# Autodesk Inventor assembly: Lift 3
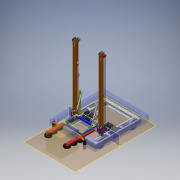
[picture p0: Inventor's stored thumbnail of the model, 180x180]
Saved by Autodesk Inventor 2017 SP1 (Build 210196100, 196)
## iProperties
Created: 2018-01-18
Part Number: Lift 3
Document SubType Name: Assembly
Designer: Ben
Mass: 9979.66 g
Surface Area: 70095.8 cm^2
Volume: 103427 cm^3
Density: 0.0964899 g/cm^3
Author: Ben
## Documents named in this file (23)
- C:\Users\Ben\Desktop\Projects\2018 Robot\Cube Lift\Lift 3.iam
- C:\Users\Ben\Desktop\Projects\2018 Robot\Cube Lift\Rail.ipt
- C:\Users\Ben\Desktop\Projects\2018 Robot\Chassis\2018_chassis.iam
- C:\Users\Ben\Desktop\Projects\2018 Robot\Cube Lift\roller bushing.iam
- C:\Users\Ben\Desktop\Projects\2018 Robot\Cube Lift\cube.ipt
- C:\Users\Ben\Desktop\Projects\2018 Robot\Cube Lift\carriage plate square 2.ipt
- C:\Users\Ben\Desktop\Projects\2018 Robot\Cube Lift\support plate 2.ipt
- C:\Users\Ben\Desktop\Projects\2018 Robot\Cube Lift\top pully bracket.ipt
- C:\Users\Ben\Desktop\Projects\2018 Robot\Cube Lift\pulley XL 1in.ipt
- C:\Users\Ben\Desktop\Projects\2018 Robot\Cube Lift\pulley XL 1.375in 2.ipt
- C:\Users\Ben\Desktop\Projects\2018 Robot\Cube Lift\first stage belt.ipt
- C:\Users\Ben\Desktop\Projects\2018 Robot\Cube Lift\upper anchor.ipt
- C:\Users\Ben\Desktop\Projects\2018 Robot\Cube Lift\top pully bracket 2.ipt
- C:\Users\Ben\Desktop\Projects\2018 Robot\Cube Lift\second stage belt 2.ipt
- C:\Users\Ben\Desktop\Projects\2018 Robot\Cube Lift\carriage plate for intake.ipt
- C:\Users\Ben\Desktop\Projects\2018 Robot\Cube Intake\Intake 2.iam
- C:\Users\Ben\Desktop\Projects\2018 Robot\Cube Lift\cylinder arm.ipt
- C:\Users\Ben\Desktop\Projects\2018 Robot\Cube Lift\cylinder body.ipt
- C:\Users\Ben\Desktop\Projects\2018 Robot\Cube Lift\cylinder piston.ipt
- C:\Users\Ben\Desktop\Projects\2018 Robot\Cube Lift\line pulley.ipt
- C:\Users\Ben\Desktop\Projects\2018 Robot\Cube Lift\outside carriage plate.ipt
- C:\Users\Ben\Desktop\Projects\2018 Robot\Cube Lift\driveshaft.ipt
- C:\Users\Ben\Desktop\Projects\2018 Robot\Cube Lift\first stage spacer.ipt
## Components (55 placed, 22 different names)
1. Rail:1 — Mate:13, Flush:15, Flush:16, Mate:20, Mate:21, Mate:22, Mate:23, Mate:30, Flush:26, Flush:27, Flush:28, Flush:29, Mate:39, Flush:30, Angle:2, Flush:33, Mate:44, Flush:43, Mate:72, Flush:53
2. 2018_chassis:1 [sub-assembly] — Mate:1, Flush:3, Flush:4, Mate:13, Flush:15, Flush:21, Flush:46, Mate:64, Flush:49, Flush:54, Mate:78
3. Rail:3 — Mate:5, Flush:16, Mate:24, Flush:34, Mate:48, Flush:35, Angle:4, Mate:50, Flush:40, Flush:41, Flush:42, Mate:54, Mate:55, Flush:64
4. roller bushing:1 [sub-assembly] — Mate:38, Flush:28
5. carriage plate square 2:1 — Mate:5, Mate:20, Mate:21, Mate:22, Mate:23, Mate:24, Mate:36, Mate:37, Mate:38, Mate:66, Mate:67, Mate:73, Mate:74
6. roller bushing:2 [sub-assembly] — Mate:36, Flush:26
7. roller bushing:3 [sub-assembly] — Mate:37, Flush:27
8. roller bushing:4 [sub-assembly] — Flush:42, Insert:11
9. roller bushing:5 [sub-assembly] — Mate:53, Flush:40
10. roller bushing:6 [sub-assembly] — Flush:41, Mate:56
11. support plate 2:1 — Mate:30, Insert:8, Flush:43, Mate:64, Flush:56, Mate:103
12. top pully bracket:1 — Flush:29, Mate:39, Flush:30, Mate:40, Flush:31, Mate:65
13. pulley XL 1in:1 — Insert:8, Insert:9
14. pulley XL 1.375in 2:1 — Mate:40, Flush:31
15. first stage belt:1 — Insert:9, Angle:2, Flush:65
16. upper anchor:1 — Flush:33, Mate:44, Mate:65
17. top pully bracket 2:1 — Flush:34, Mate:48, Flush:35, Mate:70, Mate:71
18. second stage belt 2:1 — Angle:4, Mate:68, Mate:69, Flush:66
19. carriage plate for intake:1 — Mate:50, Mate:53, Mate:54, Mate:55, Insert:11, Mate:56, Mate:57, Insert:12, Insert:16, Flush:49
20. Intake 2:1 [sub-assembly] — Flush:45, Mate:57, Insert:15, Mate:90, Insert:29
21. cylinder arm:1 — Insert:12, Mate:62, Insert:16
22. cube:2 — Mate:58, Flush:48
23. cylinder body:1 — Mate:62, Mate:63
24. cylinder piston:1 — Mate:63, Insert:15
25. line pulley:1 — Mate:66, Mate:67, Mate:68, Mate:69
26. line pulley:2 — Mate:70, Mate:71
27. outside carriage plate:1 — Mate:72, Mate:73, Mate:74
28. driveshaft:1 — Flush:52, Mate:103, Mate:104
29. support plate 2:2 — Mate:79, Flush:55, Flush:56, Insert:25, Mate:104
30. Rail:4 — Flush:57, Mate:86, Flush:58, Mate:87, Mate:88, Mate:89, Flush:59, Mate:93, Flush:60, Flush:63, Flush:64
31. Rail:5 — Flush:53, Flush:54, Mate:78, Mate:79, Flush:55, Mate:80, Mate:81, Mate:82, Flush:57, Mate:83, Mate:94, Flush:61, Flush:62, Mate:99
32. outside carriage plate:2 — Mate:80, Mate:81, Mate:82, Insert:19, Insert:20, Insert:21, Mate:84, Mate:85
33. carriage plate square 2:2 — Mate:83, Mate:84, Mate:85, Mate:86, Flush:58, Insert:26
34. carriage plate for intake:2 — Mate:87, Mate:88, Mate:89, Insert:22, Insert:23, Insert:24, Mate:90, Insert:27, Insert:28
35. roller bushing:7 [sub-assembly] — Insert:19, Insert:32
36. roller bushing:8 [sub-assembly] — Insert:20, Insert:33
37. roller bushing:9 [sub-assembly] — Insert:24
38. roller bushing:10 [sub-assembly] — Insert:21, Insert:31
39. roller bushing:11 [sub-assembly] — Insert:22
40. roller bushing:12 [sub-assembly] — Insert:23
41. pulley XL 1in:2 — Insert:25, Insert:30
42. line pulley:3 — Insert:26, Mate:101, Mate:102
43. cylinder arm:2 — Insert:27, Insert:28, Mate:92
44. cylinder body:2 — Mate:92
45. cylinder piston:2 — Insert:29
46. top pully bracket:2 — Mate:94, Flush:61, Flush:62, Mate:95, Mate:96, Mate:100
47. top pully bracket 2:2 — Flush:59, Mate:93, Flush:60, Mate:97, Mate:98
48. pulley XL 1.375in 2:2 — Mate:95, Mate:96
49. line pulley:4 — Mate:97, Mate:98
50. upper anchor:2 — Mate:99, Mate:100, Flush:63
51. first stage belt:2 — Insert:30, Flush:65
52. second stage belt 2:2 — Mate:101, Mate:102, Flush:66
53. first stage spacer:1 — Insert:31
54. first stage spacer:2 — Insert:32
55. first stage spacer:3 — Insert:33
## Relationships (126: Mate 63, Flush 40, Insert 21, Angle 2)
- Mate:1 (44.45 mm): 2018_chassis:1
- Flush:3: 2018_chassis:1
- Flush:4: 2018_chassis:1
- Mate:5: Rail:3 ↔ carriage plate square 2:1
- Mate:13: Rail:1 ↔ 2018_chassis:1
- Flush:15 (190.5 mm): Rail:1 ↔ 2018_chassis:1
- Flush:16: Rail:1 ↔ Rail:3
- Mate:20 (9.525 mm): Rail:1 ↔ carriage plate square 2:1
- Mate:21 (13.9192 mm): Rail:1 ↔ carriage plate square 2:1
- Mate:22 (13.9192 mm): Rail:1 ↔ carriage plate square 2:1
- Mate:23 (13.9192 mm): Rail:1 ↔ carriage plate square 2:1
- Mate:24: Rail:3 ↔ carriage plate square 2:1
- Flush:18 (1397 mm)
- Flush:19 (1930.4 mm)
- Flush:20 (2184.4 mm)
- Flush:21 (-508 mm): 2018_chassis:1
- Mate:30: Rail:1 ↔ support plate 2:1
- Mate:36: carriage plate square 2:1 ↔ roller bushing:2
- Flush:26 (-2.3622 mm): Rail:1 ↔ roller bushing:2
- Mate:37: carriage plate square 2:1 ↔ roller bushing:3
- Flush:27 (-2.3622 mm): Rail:1 ↔ roller bushing:3
- Mate:38: roller bushing:1 ↔ carriage plate square 2:1
- Flush:28 (2.3622 mm): Rail:1 ↔ roller bushing:1
- Flush:29 (-1.5875 mm): Rail:1 ↔ top pully bracket:1
- Mate:39: Rail:1 ↔ top pully bracket:1
- Flush:30 (6.35 mm): Rail:1 ↔ top pully bracket:1
- Insert:8 (4.7625 mm): support plate 2:1 ↔ pulley XL 1in:1
- Mate:40: top pully bracket:1 ↔ pulley XL 1.375in 2:1
- Flush:31: top pully bracket:1 ↔ pulley XL 1.375in 2:1
- Insert:9 (1.5875 mm): pulley XL 1in:1 ↔ first stage belt:1
- Angle:2 (0 deg): Rail:1 ↔ first stage belt:1
- Flush:33: Rail:1 ↔ upper anchor:1
- Mate:44: Rail:1 ↔ upper anchor:1
- Flush:34 (-1.5875 mm): Rail:3 ↔ top pully bracket 2:1
- Mate:48: Rail:3 ↔ top pully bracket 2:1
- Flush:35 (-6.35 mm): Rail:3 ↔ top pully bracket 2:1
- Angle:4 (0 deg): Rail:3 ↔ second stage belt 2:1
- Mate:50 (2.3622 mm): Rail:3 ↔ carriage plate for intake:1
- Mate:53: roller bushing:5 ↔ carriage plate for intake:1
- Flush:40 (-2.3622 mm): Rail:3 ↔ roller bushing:5
- Flush:41 (-2.3622 mm): Rail:3 ↔ roller bushing:6
- Flush:42 (-2.3622 mm): Rail:3 ↔ roller bushing:4
- Mate:54 (13.9192 mm): Rail:3 ↔ carriage plate for intake:1
- Mate:55 (13.9192 mm): Rail:3 ↔ carriage plate for intake:1
- Insert:11: roller bushing:4 ↔ carriage plate for intake:1
- Mate:56: roller bushing:6 ↔ carriage plate for intake:1
- Flush:43: Rail:1 ↔ support plate 2:1
- Flush:45: Intake 2:1
- Flush:46 (406.4 mm): 2018_chassis:1
- Mate:57: carriage plate for intake:1 ↔ Intake 2:1
- Insert:12: carriage plate for intake:1 ↔ cylinder arm:1
- Mate:58: cube:2
- Flush:48: cube:2
- Mate:62: cylinder arm:1 ↔ cylinder body:1
- Mate:63: cylinder body:1 ↔ cylinder piston:1
- Insert:15 (1.5875 mm): Intake 2:1 ↔ cylinder piston:1
- Mate:64 (-11.6078 mm): 2018_chassis:1 ↔ support plate 2:1
- Insert:16: carriage plate for intake:1 ↔ cylinder arm:1
- Flush:49 (-158.75 mm): 2018_chassis:1 ↔ carriage plate for intake:1
- Mate:65: top pully bracket:1 ↔ upper anchor:1
- Mate:66: carriage plate square 2:1 ↔ line pulley:1
- Mate:67 (3.175 mm): carriage plate square 2:1 ↔ line pulley:1
- Mate:68: second stage belt 2:1 ↔ line pulley:1
- Mate:69 (0.7937 mm): second stage belt 2:1 ↔ line pulley:1
- Mate:70: top pully bracket 2:1 ↔ line pulley:2
- Mate:71 (4.7625 mm): top pully bracket 2:1 ↔ line pulley:2
- Mate:72 (2.3622 mm): Rail:1 ↔ outside carriage plate:1
- Mate:73: carriage plate square 2:1 ↔ outside carriage plate:1
- Mate:74: carriage plate square 2:1 ↔ outside carriage plate:1
- Flush:52: driveshaft:1
- Flush:53: Rail:1 ↔ Rail:5
- Flush:54: 2018_chassis:1 ↔ Rail:5
- Mate:78: 2018_chassis:1 ↔ Rail:5
- Mate:79: support plate 2:2 ↔ Rail:5
- Flush:55: support plate 2:2 ↔ Rail:5
- Flush:56: support plate 2:1 ↔ support plate 2:2
- Mate:80 (2.3622 mm): Rail:5 ↔ outside carriage plate:2
- Mate:81 (13.9192 mm): Rail:5 ↔ outside carriage plate:2
- Mate:82 (13.9192 mm): Rail:5 ↔ outside carriage plate:2
- Insert:19: outside carriage plate:2 ↔ roller bushing:7
- Insert:20: outside carriage plate:2 ↔ roller bushing:8
- Insert:21: outside carriage plate:2 ↔ roller bushing:10
- Flush:57: Rail:4 ↔ Rail:5
- Mate:83 (9.525 mm): Rail:5 ↔ carriage plate square 2:2
- Mate:84: outside carriage plate:2 ↔ carriage plate square 2:2
- Mate:85: outside carriage plate:2 ↔ carriage plate square 2:2
- Mate:86: Rail:4 ↔ carriage plate square 2:2
- Flush:58: Rail:4 ↔ carriage plate square 2:2
- Mate:87 (2.3622 mm): Rail:4 ↔ carriage plate for intake:2
- Mate:88 (13.9192 mm): Rail:4 ↔ carriage plate for intake:2
- Mate:89 (13.9192 mm): Rail:4 ↔ carriage plate for intake:2
- Insert:22: carriage plate for intake:2 ↔ roller bushing:11
- Insert:23: carriage plate for intake:2 ↔ roller bushing:12
- Insert:24: carriage plate for intake:2 ↔ roller bushing:9
- Mate:90: Intake 2:1 ↔ carriage plate for intake:2
- Insert:25 (4.7625 mm): support plate 2:2 ↔ pulley XL 1in:2
- Insert:26 (3.175 mm): carriage plate square 2:2 ↔ line pulley:3
- Insert:27: carriage plate for intake:2 ↔ cylinder arm:2
- Insert:28: carriage plate for intake:2 ↔ cylinder arm:2
- [Mate]: cylinder body:2 ↔ cylinder piston:2
- Mate:92: cylinder arm:2 ↔ cylinder body:2
- Insert:29 (1.5875 mm): Intake 2:1 ↔ cylinder piston:2
- Flush:59 (1.5875 mm): Rail:4 ↔ top pully bracket 2:2
- Mate:93: Rail:4 ↔ top pully bracket 2:2
- Flush:60 (6.35 mm): Rail:4 ↔ top pully bracket 2:2
- Mate:94: Rail:5 ↔ top pully bracket:2
- Flush:61 (-1.5875 mm): Rail:5 ↔ top pully bracket:2
- Flush:62 (-6.35 mm): Rail:5 ↔ top pully bracket:2
- Mate:95 (6.35 mm): top pully bracket:2 ↔ pulley XL 1.375in 2:2
- Mate:96: top pully bracket:2 ↔ pulley XL 1.375in 2:2
- Mate:97: top pully bracket 2:2 ↔ line pulley:4
- Mate:98 (4.7625 mm): top pully bracket 2:2 ↔ line pulley:4
- Mate:99: Rail:5 ↔ upper anchor:2
- Mate:100: top pully bracket:2 ↔ upper anchor:2
- Flush:63: Rail:4 ↔ upper anchor:2
- Flush:64: Rail:3 ↔ Rail:4
- Insert:30 (1.5875 mm): pulley XL 1in:2 ↔ first stage belt:2
- Mate:101: line pulley:3 ↔ second stage belt 2:2
- Mate:102 (0.7937 mm): line pulley:3 ↔ second stage belt 2:2
- Flush:65: first stage belt:1 ↔ first stage belt:2
- Flush:66: second stage belt 2:1 ↔ second stage belt 2:2
- Insert:31: roller bushing:10 ↔ first stage spacer:1
- Insert:32: roller bushing:7 ↔ first stage spacer:2
- Insert:33: roller bushing:8 ↔ first stage spacer:3
- Mate:103: support plate 2:1 ↔ driveshaft:1
- Mate:104: driveshaft:1 ↔ support plate 2:2
## Named parameters: d215_d160 = 0 mm
